# Autodesk Inventor assembly: Solid1_1
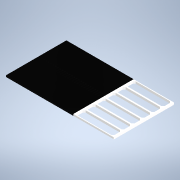
[picture p0: Inventor's stored thumbnail of the model, 180x180]
Saved by Autodesk Inventor 2020.3 (Build 243373000, 373)
## iProperties
Created: 2021-04-10
Part Number: Solid1_1
Document SubType Name: Assembly
Designer: juanp
Author: juanp
## Documents named in this file (3)
- C:\Users\juanp\Desktop\Robocol\Nuevo EVA\V1\Cajas\Solid1_1.iam
- C:\Users\juanp\Desktop\Robocol\Nuevo EVA\V1\Cajas\Solid6.ipt
- C:\Users\juanp\Desktop\Robocol\Nuevo EVA\V1\Cajas\Puerta Cremallera.ipt
## Components (2 placed, 2 different names)
1. Solid6:1 — Flush:1, Flush:2, Mate:1
2. Puerta Cremallera:1 — Flush:1, Flush:2, Mate:1
## Relationships (3: Flush 2, Mate 1)
- Flush:1: Solid6:1 ↔ Puerta Cremallera:1
- Flush:2: Solid6:1 ↔ Puerta Cremallera:1
- Mate:1: Solid6:1 ↔ Puerta Cremallera:1
